# Autodesk Inventor assembly: guide_servo
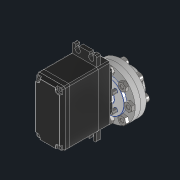
[picture p0: Inventor's stored thumbnail of the model, 180x180]
Saved by Autodesk Inventor 2022 (Build 260153000, 153)
## iProperties
Created: 2021-08-27
Part Number: guide_servo
Document SubType Name: Assembly
Designer: Yuta Kage
Author: Yuta Kage
## Documents named in this file (7)
- C:\Users\yuta0\Documents\GitHub\catchrobo_hardware\assy-shooter\guide_servo.iam
- C:\Users\yuta0\Documents\GitHub\catchrobo_hardware\assy-robot\MG_996R.iam
- C:\Users\yuta0\Documents\GitHub\catchrobo_hardware\assy-shooter\s_base5.ipt
- C:\Users\yuta0\Documents\GitHub\catchrobo_hardware\assy-robot\CB3-10.ipt
- C:\Users\yuta0\Documents\GitHub\catchrobo_hardware\assy-shooter\s_base6.ipt
- C:\Users\yuta0\Documents\GitHub\catchrobo_hardware\assy-shooter\SCSTR6-8.iam
- C:\Users\yuta0\Documents\GitHub\catchrobo_hardware\assy-robot\LBNR3.ipt
## Components (28 placed, 6 different names)
1. MG_996R:1 [sub-assembly] — メイト:1, メイト:2, メイト:3
2. s_base5:1 — メイト:1, メイト:2, メイト:3, メイト:4, メイト:5, メイト:9, メイト:13, メイト:14, メイト:15
3. s_base6:1 — メイト:6, メイト:7, メイト:8, メイト:9, メイト:10, メイト:11, メイト:12, メイト:13, メイト:16, メイト:17
4. SCSTR6-8:1 [sub-assembly] — メイト:6, メイト:7, メイト:8
5. CB3-10:1 — メイト:4, メイト:5
6. CB3-10:5 — メイト:11, メイト:12
7. CB3-10:2
8. CB3-10:6
9. CB3-10:3
10. CB3-10:7
11. CB3-10:4 — メイト:10
12. CB3-10:8
13. LBNR3:1 — メイト:14, メイト:15
14. CB3-10:9 — メイト:16, メイト:17
15. LBNR3:2
16. CB3-10:10
17. LBNR3:3
18. CB3-10:11
19. LBNR3:4
20. CB3-10:12
21. LBNR3:5
22. CB3-10:13
23. LBNR3:6
24. CB3-10:14
25. LBNR3:7
26. CB3-10:15
27. LBNR3:8
28. CB3-10:16
## Component patterns: (4 elements, first: CB3-10:1 + CB3-10:5), (8 elements, first: LBNR3:1 + CB3-10:9)
## Relationships (17: Mate 17)
- メイト:1 [Mate]: MG_996R:1 ↔ s_base5:1
- メイト:2 [Mate]: MG_996R:1 ↔ s_base5:1
- メイト:3 [Mate]: MG_996R:1 ↔ s_base5:1
- メイト:4 [Mate]: s_base5:1 ↔ CB3-10:1
- メイト:5 [Mate]: s_base5:1 ↔ CB3-10:1
- メイト:6 [Mate]: s_base6:1 ↔ SCSTR6-8:1
- メイト:7 [Mate]: s_base6:1 ↔ SCSTR6-8:1
- メイト:8 [Mate]: s_base6:1 ↔ SCSTR6-8:1
- メイト:9 [Mate]: s_base5:1 ↔ s_base6:1
- メイト:10 [Mate]: s_base6:1 ↔ CB3-10:4
- メイト:11 [Mate]: s_base6:1 ↔ CB3-10:5
- メイト:12 [Mate]: s_base6:1 ↔ CB3-10:5
- メイト:13 [Mate]: s_base5:1 ↔ s_base6:1
- メイト:14 [Mate]: s_base5:1 ↔ LBNR3:1
- メイト:15 [Mate]: s_base5:1 ↔ LBNR3:1
- メイト:16 [Mate]: s_base6:1 ↔ CB3-10:9
- メイト:17 [Mate]: s_base6:1 ↔ CB3-10:9
